# Autodesk Inventor assembly: sub-frame
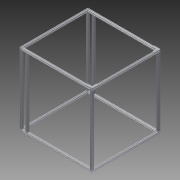
[picture p0: Inventor's stored thumbnail of the model, 180x180]
Saved by Autodesk Inventor 2013 (Build 170138000, 138)
## iProperties
Created: 2013-09-17
Part Number: sub-frame
Document SubType Name: Assembly
Designer: Ian
Author: Ian
## Documents named in this file (3)
- C:\Users\Ian\Documents\Inventor\xyPartStorage\loader\sub-frame.iam
- C:\Users\Ian\Documents\Inventor\xyPartStorage\80-20 models\T-slot\1515-48.ipt
- C:\Users\Ian\Documents\Inventor\xyPartStorage\angle-90-plate.ipt
## Components (16 placed, 2 different names)
1. 1515-48:1 — Flush:31, Flush:32, Flush:33, Flush:36
2. 1515-48:2 — Flush:31, Flush:35, Flush:37
3. 1515-48:3 — Flush:32, Flush:34, Flush:38
4. 1515-48:4
5. angle-90-plate:1
6. angle-90-plate:2
7. 1515-48:5 — Flush:38, Mate:20, Flush:39
8. 1515-48:6 — Flush:37, Flush:39
9. 1515-48:7
10. 1515-48:8
11. 1515-48:9
12. 1515-48:10
13. 1515-48:11
14. 1515-48:12
15. 1515-48:13 — Flush:35, Flush:36
16. 1515-48:14 — Flush:33, Flush:34, Mate:20
## Relationships (51: Flush 35, Mate 16)
- [Mate]: 1515-48:1 ↔ 1515-48:3
- [Flush]: 1515-48:1 ↔ 1515-48:3
- [Mate]: 1515-48:1 ↔ 1515-48:2
- [Flush]: 1515-48:1 ↔ 1515-48:2
- [Mate]: 1515-48:2 ↔ angle-90-plate:1
- [Flush]: 1515-48:2 ↔ angle-90-plate:1
- [Flush]: 1515-48:3 ↔ angle-90-plate:2
- [Mate]: 1515-48:3 ↔ angle-90-plate:2
- [Mate]: 1515-48:4 ↔ angle-90-plate:1
- [Mate]: 1515-48:2 ↔ 1515-48:4
- [Flush]: 1515-48:2 ↔ 1515-48:4
- [Flush]: 1515-48:4 ↔ angle-90-plate:1
- [Flush]: 1515-48:4 ↔ angle-90-plate:2
- [Mate]: 1515-48:3 ↔ 1515-48:7
- [Mate]: 1515-48:1 ↔ 1515-48:6
- [Mate]: 1515-48:4 ↔ 1515-48:8
- [Mate]: 1515-48:3 ↔ 1515-48:5
- [Flush]: 1515-48:4 ↔ 1515-48:7
- [Flush]: 1515-48:4 ↔ 1515-48:7
- [Flush]: 1515-48:4 ↔ 1515-48:8
- [Flush]: 1515-48:1 ↔ 1515-48:5
- [Flush]: 1515-48:4 ↔ 1515-48:8
- [Flush]: 1515-48:1 ↔ 1515-48:6
- [Mate]: 1515-48:7 ↔ 1515-48:11
- [Flush]: 1515-48:7 ↔ 1515-48:11
- [Flush]: 1515-48:7 ↔ 1515-48:11
- [Flush]: 1515-48:9 ↔ 1515-48:11
- [Mate]: 1515-48:9 ↔ 1515-48:11
- [Flush]: 1515-48:9 ↔ 1515-48:11
- [Flush]: 1515-48:9 ↔ 1515-48:12
- [Flush]: 1515-48:5 ↔ 1515-48:12
- [Flush]: 1515-48:10 ↔ 1515-48:12
- [Mate]: 1515-48:10 ↔ 1515-48:12
- [Flush]: 1515-48:10 ↔ 1515-48:12
- [Flush]: 1515-48:1 ↔ 1515-48:12
- [Flush]: 1515-48:1 ↔ 1515-48:12
- [Flush]: 1515-48:9 ↔ 1515-48:12
- [Mate]: 1515-48:3 ↔ 1515-48:14
- [Flush]: 1515-48:1 ↔ 1515-48:14
- [Mate]: 1515-48:1 ↔ 1515-48:13
- [Flush]: 1515-48:2 ↔ 1515-48:13
- Flush:31: 1515-48:1 ↔ 1515-48:2
- Flush:32: 1515-48:1 ↔ 1515-48:3
- Flush:33: 1515-48:1 ↔ 1515-48:14
- Flush:34: 1515-48:3 ↔ 1515-48:14
- Flush:35: 1515-48:2 ↔ 1515-48:13
- Flush:36: 1515-48:1 ↔ 1515-48:13
- Flush:37: 1515-48:2 ↔ 1515-48:6
- Flush:38: 1515-48:3 ↔ 1515-48:5
- Mate:20 (62.992 mm): 1515-48:5 ↔ 1515-48:14
- Flush:39: 1515-48:5 ↔ 1515-48:6
